# Autodesk Inventor assembly: Axle With single sprocket
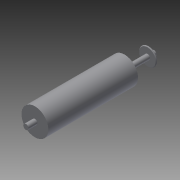
[picture p0: Inventor's stored thumbnail of the model, 180x180]
Saved by Autodesk Inventor 2015 (Build 190159000, 159)
## iProperties
Created: 2015-01-11
Part Number: Axle With single sprocket
Document SubType Name: Assembly
Designer: chapale16
Author: chapale16
## Documents named in this file (3)
- \\lhssvr02\Homedirs\Robotics Club\CAD Model 2015\Box Beam Drive Base\Axle With single sprocket.iam
- \\lhssvr02\Homedirs\Robotics Club\CAD Model 2015\Box Beam Drive Base\Sprocket Large_MIR.ipt
- \\lhssvr02\Homedirs\Robotics Club\CAD Model 2015\Box Beam Drive Base\Conveyor Axle.ipt
## Components (2 placed, 2 different names)
1. Sprocket Large_MIR:1 — Mate:1
2. Conveyor Axle:1 — Mate:1
## Relationships (1: Mate 1)
- Mate:1: Sprocket Large_MIR:1 ↔ Conveyor Axle:1
